# Autodesk Inventor assembly: hang support
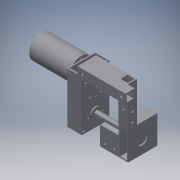
[picture p0: Inventor's stored thumbnail of the model, 180x180]
Saved by Autodesk Inventor 2016 (Build 200138000, 138)
## iProperties
Created: 2016-04-20
Part Number: hang support
Document SubType Name: Assembly
Designer: gus
Author: gus
## Documents named in this file (9)
- \\Mac\Home\Desktop\1510-stronghold-CAD-master\hang arm 2.0\hang support.iam
- \\Mac\Home\Desktop\1510-stronghold-CAD-master\hang arm 2.0\support block.ipt
- \\Mac\Home\Desktop\1510-stronghold-CAD-master\hang arm 2.0\support block 2.ipt
- \\Mac\Home\Desktop\1510-stronghold-CAD-master\hang arm 2.0\upright beam.ipt
- \\Mac\Home\Desktop\1510-stronghold-CAD-master\hang arm 2.0\gusset.ipt
- \\Mac\Home\Desktop\1510-stronghold-CAD-master\hang arm 2.0\other end support.ipt
- \\Mac\Home\Desktop\1510-stronghold-CAD-master\hang arm 2.0\angle gusset.ipt
- \\Mac\Home\Desktop\1510-stronghold-CAD-master\hang arm 2.0\tb nano\Toughbox+Nano+All+Shafts+v2-2.ipt
- \\Mac\Home\Desktop\1510-stronghold-CAD-master\hang arm 2.0\bottom gusset.ipt
## Components (9 placed, 8 different names)
1. support block:3 — Mate:7, Flush:31, Flush:32, Mate:9, Flush:33
2. upright beam:1 — Flush:16, Mate:6, Mate:8, Mate:9, Flush:33, Flush:34, Mate:13, Flush:38, Flush:39, Flush:41, Flush:42
3. other end support:1 — Flush:16, Flush:20, Flush:23, Flush:24, Mate:6, Flush:30, Mate:10, Mate:11, Flush:43
4. angle gusset:1 — Flush:20, Flush:21, Flush:23, Flush:24
5. Toughbox+Nano+All+Shafts+v2-2:1 — Flush:21, Flush:30
6. support block 2:1 — Mate:7, Flush:31, Flush:32, Mate:8, Flush:40
7. gusset:1 — Mate:13, Flush:38, Flush:39
8. gusset:3 — Mate:10, Flush:34, Mate:11, Flush:43
9. bottom gusset:1 — Flush:40, Flush:41, Flush:42
## Relationships (23: Flush 16, Mate 7)
- Flush:16: upright beam:1 ↔ other end support:1
- Flush:20: other end support:1 ↔ angle gusset:1
- Flush:21: angle gusset:1 ↔ Toughbox+Nano+All+Shafts+v2-2:1
- Flush:23: other end support:1 ↔ angle gusset:1
- Flush:24: other end support:1 ↔ angle gusset:1
- Mate:6: upright beam:1 ↔ other end support:1
- Flush:30: other end support:1 ↔ Toughbox+Nano+All+Shafts+v2-2:1
- Mate:7: support block:3 ↔ support block 2:1
- Flush:31: support block:3 ↔ support block 2:1
- Flush:32: support block:3 ↔ support block 2:1
- Mate:8: upright beam:1 ↔ support block 2:1
- Mate:9: support block:3 ↔ upright beam:1
- Flush:33: support block:3 ↔ upright beam:1
- Mate:10: other end support:1 ↔ gusset:3
- Flush:34: upright beam:1 ↔ gusset:3
- Mate:11 (-25.4 mm): other end support:1 ↔ gusset:3
- Mate:13: upright beam:1 ↔ gusset:1
- Flush:38: upright beam:1 ↔ gusset:1
- Flush:39 (-25.4 mm): upright beam:1 ↔ gusset:1
- Flush:40: support block 2:1 ↔ bottom gusset:1
- Flush:41: upright beam:1 ↔ bottom gusset:1
- Flush:42: upright beam:1 ↔ bottom gusset:1
- Flush:43: other end support:1 ↔ gusset:3
